# Autodesk Inventor assembly: Podnóżek
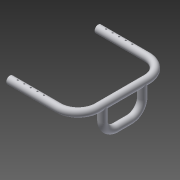
[picture p0: Inventor's stored thumbnail of the model, 180x180]
Saved by Autodesk Inventor 2014 SP2 (Build 180246200, 246)
## iProperties
Created: 2016-01-13
Part Number: Podnóżek
Document SubType Name: Konstrukcja spawana
Designer: graaapsik
Weld Material: Aluminium AW-7020
Author: graaapsik
## Documents named in this file (6)
- G:\Dokumenty\♥ MECHANIKA\2 semestr\ZSW CAD CAM CAE\Projekt\Model\Podnóżek.iam
- G:\Dokumenty\♥ MECHANIKA\2 semestr\ZSW CAD CAM CAE\Projekt\Model\Rura_pionowa_podnóżka.ipt
- G:\Dokumenty\♥ MECHANIKA\2 semestr\ZSW CAD CAM CAE\Projekt\Model\Rura_pozioma_podnóżka.ipt
- G:\Dokumenty\♥ MECHANIKA\2 semestr\ZSW CAD CAM CAE\Projekt\Model\ISO 7092 - ST 6 - 140 HV.ipt
- G:\Dokumenty\♥ MECHANIKA\2 semestr\ZSW CAD CAM CAE\Projekt\Model\ISO 4035 - M6ISO.ipt
- G:\Dokumenty\♥ MECHANIKA\2 semestr\ZSW CAD CAM CAE\Projekt\Model\ISO 4016 - M6 x 40.ipt
## Components (10 placed, 5 different names)
1. Rura_pionowa_podnóżka:1 — Równoległy:2, Zestawiający:1, Równoległy:3, Styczny:1, Styczny:2, Styczny:3, Styczny:4, Zestawiający:14
2. Rura_pozioma_podnóżka:1 — Równoległy:2, Zestawiający:1, Równoległy:3
3. ISO 7092 ST 6 - 140 HV:1 — Styczny:2
4. ISO 7092 ST 6 - 140 HV:2 — Styczny:1, Zestawiający:14, Wstaw:2
5. ISO 7092 ST 6 - 140 HV:3 — Styczny:3, Wstaw:1
6. ISO 7092 ST 6 - 140 HV:4 — Styczny:4
7. ISO 4035 M6:1
8. ISO 4035 M6:2
9. ISO 4016 M6 x 40:3 — Wstaw:1
10. ISO 4016 M6 x 40:4 — Wstaw:2
## Relationships (12: Mate 4, Tangent 4, Flush 2, Insert 2)
- Równoległy:2 [Flush]: Rura_pionowa_podnóżka:1 ↔ Rura_pozioma_podnóżka:1
- Zestawiający:1 [Mate] (-0.1 mm): Rura_pionowa_podnóżka:1 ↔ Rura_pozioma_podnóżka:1
- Równoległy:3 [Flush]: Rura_pionowa_podnóżka:1 ↔ Rura_pozioma_podnóżka:1
- Styczny:1 [Tangent] (2.5 mm): Rura_pionowa_podnóżka:1 ↔ ISO 7092 ST 6 - 140 HV:2
- Styczny:2 [Tangent] (2.5 mm): Rura_pionowa_podnóżka:1 ↔ ISO 7092 ST 6 - 140 HV:1
- [Mate]: ISO 7092 ST 6 - 140 HV:1 ↔ ISO 4035 M6:1
- Styczny:3 [Tangent] (2.5 mm): Rura_pionowa_podnóżka:1 ↔ ISO 7092 ST 6 - 140 HV:3
- Styczny:4 [Tangent] (2.5 mm): Rura_pionowa_podnóżka:1 ↔ ISO 7092 ST 6 - 140 HV:4
- [Mate]: ISO 7092 ST 6 - 140 HV:4 ↔ ISO 4035 M6:2
- Zestawiający:14 [Mate]: Rura_pionowa_podnóżka:1 ↔ ISO 7092 ST 6 - 140 HV:2
- Wstaw:1 [Insert]: ISO 7092 ST 6 - 140 HV:3 ↔ ISO 4016 M6 x 40:3
- Wstaw:2 [Insert]: ISO 7092 ST 6 - 140 HV:2 ↔ ISO 4016 M6 x 40:4
